# Autodesk Inventor assembly: Mold Design1
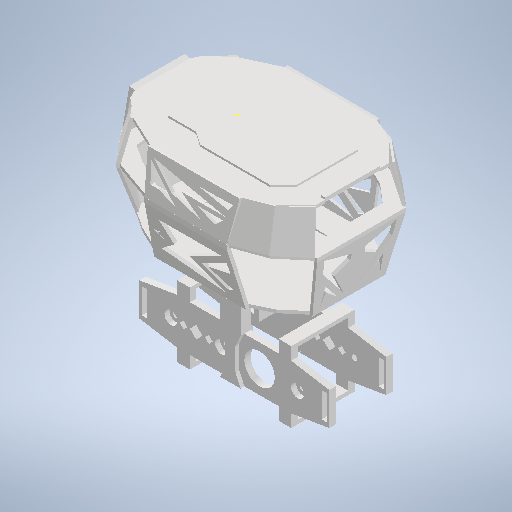
[picture p0: Inventor's stored thumbnail of the model, 512x512]
Saved by Autodesk Inventor 2025.2 (Build 292293000, 293)
## iProperties
Created: 2025-04-15
Part Number: Mold Design1
Document SubType Name: Assembly
Designer: ziyuz
Author: ziyuz
## Documents named in this file (11)
- F:\autoeskinvetersave\lanche\Mold Design1.iam
- F:\autoeskinvetersave\lanche\Part1EDDV4.ipt
- F:\autoeskinvetersave\lanche\Part2EDD.ipt
- F:\autoeskinvetersave\lanche\Part3EDD.ipt
- F:\autoeskinvetersave\lanche\Part4EDD.ipt
- F:\autoeskinvetersave\lanche\Part6.ipt
- F:\autoeskinvetersave\lanchetop\Connecting pt.1.ipt
- F:\autoeskinvetersave\lanchetop\Connecting pt.2.ipt
- F:\autoeskinvetersave\lanchetop\Side w motor.ipt
- F:\autoeskinvetersave\lanchetop\SideV1.ipt
- F:\autoeskinvetersave\Part3.ipt
## Components (14 placed, 10 different names)
1. Part1EDDV4:1 — Rigid:1, Rotational:1, Rotational:2, Rotational:3, Mate:1, Mate:2, Mate:3
2. Part2EDD:1 — Rigid:1
3. Part3EDD:1 — Rotational:2
4. Part3EDD:2 — Rotational:3
5. Part4EDD:1 — Rotational:1, Mate:8, Mate:9
6. Part6:1 — Mate:1, Mate:2, Mate:3
7. Connecting pt.1:1 — Mate:4, Mate:5, Flush:1, Mate:8, Mate:9, Rigid:2
8. Connecting pt.2:1 — Mate:6, Mate:7, Flush:2, Rigid:2
9. Side w motor:1 — Mate:6, Mate:7, Flush:2, Mate:10, Mate:15, Flush:5, Mate:16, Flush:6, Mate:17
10. SideV1:2 — Mate:4, Mate:5, Flush:1, Flush:3, Mate:11, Mate:12, Mate:13, Flush:4, Mate:14
11. Part3:1 — Mate:10, Flush:3, Mate:11, Mate:12
12. Part3:2 — Mate:13, Flush:4, Mate:14
13. Part3:3 — Mate:15, Flush:5
14. Part3:4 — Mate:16, Flush:6, Mate:17
## Relationships (28: Mate 17, Flush 6, RevoluteJoint 3, WeldJoint 2)
- Rigid:1 [WeldJoint] (12.5 mm): Part1EDDV4:1 ↔ Part2EDD:1
- Rotational:1 [RevoluteJoint] (-0.5 mm): Part1EDDV4:1 ↔ Part4EDD:1
- Rotational:2 [RevoluteJoint]: Part1EDDV4:1 ↔ Part3EDD:1
- Rotational:3 [RevoluteJoint]: Part1EDDV4:1 ↔ Part3EDD:2
- Mate:1: Part1EDDV4:1 ↔ Part6:1
- Mate:2: Part1EDDV4:1 ↔ Part6:1
- Mate:3: Part1EDDV4:1 ↔ Part6:1
- Mate:4: Connecting pt.1:1 ↔ SideV1:2
- Mate:5: Connecting pt.1:1 ↔ SideV1:2
- Flush:1: Connecting pt.1:1 ↔ SideV1:2
- Mate:6: Connecting pt.2:1 ↔ Side w motor:1
- Mate:7: Connecting pt.2:1 ↔ Side w motor:1
- Flush:2: Connecting pt.2:1 ↔ Side w motor:1
- Mate:8: Part4EDD:1 ↔ Connecting pt.1:1
- Mate:9: Part4EDD:1 ↔ Connecting pt.1:1
- Rigid:2 [WeldJoint]: Connecting pt.1:1 ↔ Connecting pt.2:1
- Mate:10: Side w motor:1 ↔ Part3:1
- Flush:3: SideV1:2 ↔ Part3:1
- Mate:11: SideV1:2 ↔ Part3:1
- Mate:12: SideV1:2 ↔ Part3:1
- Mate:13: SideV1:2 ↔ Part3:2
- Flush:4: SideV1:2 ↔ Part3:2
- Mate:14: SideV1:2 ↔ Part3:2
- Mate:15: Side w motor:1 ↔ Part3:3
- Flush:5: Side w motor:1 ↔ Part3:3
- Mate:16: Side w motor:1 ↔ Part3:4
- Flush:6: Side w motor:1 ↔ Part3:4
- Mate:17: Side w motor:1 ↔ Part3:4
